# Autodesk Inventor assembly: XM540_NO_BACK
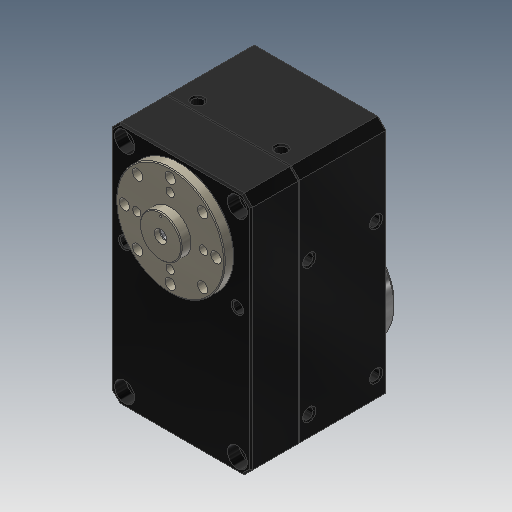
[picture p0: Inventor's stored thumbnail of the model, 512x512]
Saved by Autodesk Inventor 2019.4 (Build 234330000, 330)
## iProperties
Created: 2019-10-19
Part Number: XM540_NO_BACK
Material: 一般
Document SubType Name: Assembly
Designer: y6tada
Author: y6tada
## Documents named in this file (4)
- C:\Workspace\Yuni8\Libs\DYNAMIXEL\XM540\XM540_NO_BACK.iam
- C:\Workspace\Yuni8\Libs\DYNAMIXEL\XM540\XM540_HOUSING_TOP.ipt
- C:\Workspace\Yuni8\Libs\DYNAMIXEL\XM540\XM540_HOUSING_MIDDLE.ipt
- C:\Workspace\Yuni8\Libs\DYNAMIXEL\XM540\XM540_HORN.ipt
## Components (3 placed, 3 different names)
1. XM540_HOUSING_TOP:1 — メイト:1, メイト:2, メイト:3, メイト:4, メイト:5, フラッシュ:1
2. XM540_HOUSING_MIDDLE:1 — メイト:1, メイト:2, メイト:3
3. XM540_HORN:1 — メイト:4, メイト:5, フラッシュ:1
## Relationships (6: Mate 5, Flush 1)
- メイト:1 [Mate]: XM540_HOUSING_TOP:1 ↔ XM540_HOUSING_MIDDLE:1
- メイト:2 [Mate]: XM540_HOUSING_TOP:1 ↔ XM540_HOUSING_MIDDLE:1
- メイト:3 [Mate]: XM540_HOUSING_TOP:1 ↔ XM540_HOUSING_MIDDLE:1
- メイト:4 [Mate]: XM540_HOUSING_TOP:1 ↔ XM540_HORN:1
- メイト:5 [Mate]: XM540_HOUSING_TOP:1 ↔ XM540_HORN:1
- フラッシュ:1 [Flush]: XM540_HOUSING_TOP:1 ↔ XM540_HORN:1
